# Autodesk Inventor assembly: RC Car
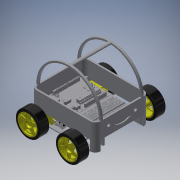
[picture p0: Inventor's stored thumbnail of the model, 180x180]
Saved by Autodesk Inventor 2019 (Build 230136000, 136)
## iProperties
Created: 2020-12-04
Part Number: RC Car
Document SubType Name: Assembly
Designer: melis
Author: melis
## Documents named in this file (7)
- C:\Users\melis\OneDrive\Desktop\Code&Mech\InventorParts\RC Car.iam
- C:\Users\melis\OneDrive\Desktop\Code&Mech\InventorParts\rc car inards\breadboard_350_pos_asm.ipt
- C:\Users\melis\OneDrive\Desktop\Code&Mech\InventorParts\rc car inards\Arduino Uno.ipt
- C:\Users\melis\Downloads\dc-gear-motor-1.snapshot.1\Model 302 DC Gearmotor.ipt
- C:\Users\melis\OneDrive\Desktop\Code&Mech\InventorParts\rc car inards\motor.ipt
- C:\Users\melis\OneDrive\Desktop\Code&Mech\InventorParts\chassis.ipt
- C:\Users\melis\OneDrive\Desktop\Code&Mech\InventorParts\rc car inards\velg.ipt
## Components (10 placed, 6 different names)
1. breadboard_350_pos_asm:1 — Mate:6
2. Arduino Uno:1 — Tangent:1, Mate:5
3. Model 302 DC Gearmotor:3 — Tangent:1
4. motor:2 — Mate:3, Mate:4, Rigid:2, Mate:13
5. motor:4 — Mate:9, Mate:10, Rigid:3, Mate:15
6. chassis:1 — Mate:3, Mate:4, Mate:5, Mate:6, Mate:9, Mate:10, Mate:13, Mate:15, Rigid:4, Rigid:5
7. velg:1 — Rigid:2
8. velg:2 — Rigid:3
9. velg:3 — Rigid:4
10. velg:4 — Rigid:5
## Relationships (13: Mate 8, WeldJoint 4, Tangent 1)
- Tangent:1: Arduino Uno:1 ↔ Model 302 DC Gearmotor:3
- Mate:3: motor:2 ↔ chassis:1
- Mate:4: motor:2 ↔ chassis:1
- Rigid:2 [WeldJoint]: motor:2 ↔ velg:1
- Mate:5: Arduino Uno:1 ↔ chassis:1
- Mate:6: breadboard_350_pos_asm:1 ↔ chassis:1
- Mate:9: motor:4 ↔ chassis:1
- Mate:10: motor:4 ↔ chassis:1
- Rigid:3 [WeldJoint]: motor:4 ↔ velg:2
- Mate:13: motor:2 ↔ chassis:1
- Mate:15: motor:4 ↔ chassis:1
- Rigid:4 [WeldJoint]: chassis:1 ↔ velg:3
- Rigid:5 [WeldJoint]: chassis:1 ↔ velg:4
